# Autodesk Inventor assembly: Assembly1
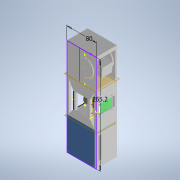
[picture p0: Inventor's stored thumbnail of the model, 180x180]
Saved by Autodesk Inventor 2022 (Build 260153000, 153)
## iProperties
Created: 2022-04-28
Part Number: Assembly1
Document SubType Name: Assembly
Designer: Oana
Author: Oana
## Documents named in this file (6)
- C:\Users\Miss Oana\Desktop\Assembly1.iam
- C:\Users\Miss Oana\Desktop\Part1.ipt
- C:\Users\Miss Oana\Desktop\New folder (2)\Scanner3D\Camera.iam
- C:\Users\Miss Oana\Desktop\New folder (2)\Scanner3D\RaspberryPi4.ipt
- C:\Users\Miss Oana\Desktop\Part2.ipt
- C:\Users\Miss Oana\Desktop\New folder (2)\Scanner3D\sevo prins xu laser.iam
## Components (5 placed, 5 different names)
1. Part1:1 — Mate:5, Mate:6, Mate:7, Mate:8, Mate:9, Mate:10, Flush:14, Flush:15, Rotational:1
2. Part2:1 — Mate:5, Mate:6, Mate:7
3. RaspberryPi4:1 — Mate:8, Mate:9, Mate:10
4. Camera:1 [sub-assembly] — Flush:14
5. sevo prins xu laser:1 [sub-assembly] — Rotational:1
## Relationships (9: Mate 6, Flush 2, RevoluteJoint 1)
- Mate:5: Part1:1 ↔ Part2:1
- Mate:6: Part1:1 ↔ Part2:1
- Mate:7: Part1:1 ↔ Part2:1
- Mate:8: Part1:1 ↔ RaspberryPi4:1
- Mate:9: Part1:1 ↔ RaspberryPi4:1
- Mate:10 (4 mm): Part1:1 ↔ RaspberryPi4:1
- Flush:14: Part1:1 ↔ Camera:1
- Flush:15: Part1:1
- Rotational:1 [RevoluteJoint] (-12 mm): Part1:1 ↔ sevo prins xu laser:1
